# Autodesk Inventor assembly: ASY дренаж угольные
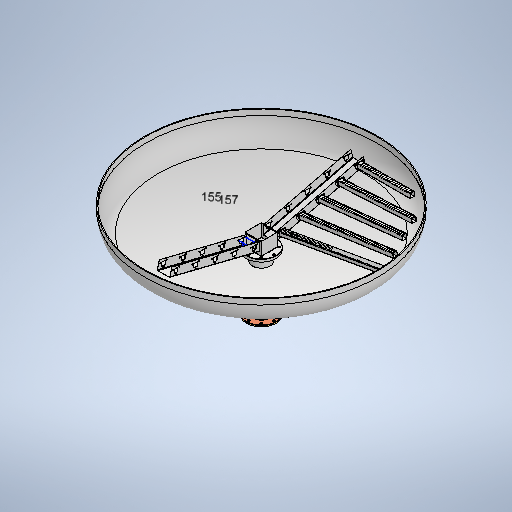
[picture p0: Inventor's stored thumbnail of the model, 512x512]
Saved by Autodesk Inventor 2025 (Build 290162010, 162A)
## iProperties
Created: 2024-12-09
Part Number: ASY дренаж угольные
Document SubType Name: Assembly
Designer: user
Author: user
## Documents named in this file (21)
- C:\Users\pokla\Documents\Inventor\Отстойник осветлитель\Manturovo_Se-clar-Gleb\Дренаж на угольные\ASY дренаж угольные.iam
- C:\Users\pokla\Documents\Inventor\Отстойник осветлитель\Manturovo_Se-clar-Gleb\Дренаж на угольные\Main filter Flange.ipt
- C:\Users\pokla\Documents\Inventor\Отстойник осветлитель\Manturovo_Se-clar-Gleb\Дренаж на угольные\drain flange.ipt
- C:\Users\pokla\Documents\Inventor\Отстойник осветлитель\Manturovo_Se-clar-Gleb\Дренаж на угольные\Part9.ipt
- C:\Users\pokla\Documents\Inventor\Отстойник осветлитель\Manturovo_Se-clar-Gleb\Дренаж на угольные\drain bottom plate.ipt
- C:\Users\pokla\Documents\Inventor\Отстойник осветлитель\Manturovo_Se-clar-Gleb\Дренаж на угольные\drain wall with flange.ipt
- C:\Users\user\YandexDisk-badmisterfox\домашниий пк\Inventor\Manturovo\Content Center Files\en-US\DIN 933\DIN 933 - M12  x 35.ipt
- C:\Users\pokla\Documents\Inventor\Отстойник осветлитель\Manturovo_Se-clar-Gleb\Дренаж на угольные\drain cup.ipt
- C:\Users\pokla\Documents\Inventor\Отстойник осветлитель\Manturovo_Se-clar-Gleb\Дренаж на угольные\Фильтр напорный угольный 30 куб час.ipt
- C:\Users\pokla\Documents\Inventor\Отстойник осветлитель\Manturovo_Se-clar-Gleb\Дренаж на угольные\MNT-CDF-301 beam 1.ipt
- C:\Users\pokla\Documents\Inventor\Отстойник осветлитель\Manturovo_Se-clar-Gleb\Дренаж на угольные\MNT-CDF-401 roof 1.ipt
- C:\Users\pokla\Documents\Inventor\Отстойник осветлитель\Manturovo_Se-clar-Gleb\Дренаж на угольные\MNT-CDF-501 box.ipt
- C:\Users\pokla\Documents\Inventor\Отстойник осветлитель\Manturovo_Se-clar-Gleb\Дренаж на угольные\MNT-CDF-502 tube.ipt
- C:\Users\pokla\Documents\Inventor\Отстойник осветлитель\Manturovo_Se-clar-Gleb\Дренаж на угольные\MNT-CDF-503  main tube 1.ipt
- C:\Users\user\YandexDisk-badmisterfox\домашниий пк\Inventor\Manturovo\Content Center Files\en-US\DIN 933\DIN 933 - M8  x 20.ipt
- C:\Users\pokla\Documents\Inventor\Отстойник осветлитель\Manturovo_Se-clar-Gleb\Дренаж на угольные\MNT-CDF-504 small tube flange.ipt
- C:\Users\pokla\Documents\Inventor\Отстойник осветлитель\Manturovo_Se-clar-Gleb\Дренаж на угольные\MNT-CDF-315 beam 5.ipt
- C:\Users\pokla\Documents\Inventor\Отстойник осветлитель\Manturovo_Se-clar-Gleb\Дренаж на угольные\MNT-CDF-312 beam 2.ipt
- C:\Users\pokla\Documents\Inventor\Отстойник осветлитель\Manturovo_Se-clar-Gleb\Дренаж на угольные\MNT-CDF-313 beam 3.ipt
- C:\Users\pokla\Documents\Inventor\Отстойник осветлитель\Manturovo_Se-clar-Gleb\Дренаж на угольные\MNT-CDF-314 beam 4.ipt
- C:\Users\pokla\Documents\Inventor\NDM-VOS_powder_hopper\Workspaces\Workspace\Cone\MNT-CDF-601 CAP.ipt
## Components (39 placed, 20 different names)
1. Main filter Flange.ipt:1 — Rigid:1
2. drain flange.ipt:1 — Rigid:1, Rigid:7
3. Part9.ipt:1 — Rigid:4, Rigid:7
4. drain bottom plate.ipt:1 — Rigid:4, Rigid:5, Rigid:6
5. drain wall with flange:1 — Rigid:3, Rigid:6, Mate:2, Flush:1, Rotational:2, Rotational:3, Rotational:4
6. DIN 933 - replaced by DIN EN 24017 M12  x 35:1 — Rigid:3
7. drain wall with flange:2 — Rigid:5, Mate:1, Rotational:1
8. DIN 933 - replaced by DIN EN 24017 M12  x 35:2 — Rotational:1
9. DIN 933 - replaced by DIN EN 24017 M12  x 35:3 — Rotational:3
10. Part1:3 — Mate:1, Mate:2, Flush:1, Rotational:5, Rotational:6
11. DIN 933 - replaced by DIN EN 24017 M12  x 35:4 — Rotational:2
12. DIN 933 - replaced by DIN EN 24017 M12  x 35:5 — Rotational:4
13. DIN 933 - replaced by DIN EN 24017 M12  x 35:6 — Rotational:6
14. DIN 933 - replaced by DIN EN 24017 M12  x 35:7 — Rotational:5
15. Фильтр напорный угольный 30 куб час:1 — Mate:4, Flush:3, Flush:4, Rigid:12
16. MNT-CDF-301 beam 1:1 — Flush:2, Mate:8, Flush:9, Rigid:22
17. MNT-CDF-401 roof 1:1 — Flush:2, Mate:8, Flush:9
18. MNT-CDF-501 box:1 — Rotational:9, Flush:8, Mate:9, Mate:10, Rotational:10, Rotational:11
19. drain flange:2 — Rigid:12, Mate:5
20. MNT-CDF-502 tube:4 — Rotational:11
21. MNT-CDF-502 tube:3 — Rotational:10
22. MNT-CDF-502 tube:2 — Rotational:9
23. MNT-CDF-503  main tube 1:1 — Rigid:14, Rigid:15
24. MNT-CDF-503  main tube 1:2 — Rigid:14, Mate:5, Mate:6, Mate:9, Mate:10
25. MNT-CDF-501 box:2 — Rigid:15, Rigid:18, Rigid:19, Rigid:20, Rigid:23, Rigid:24, Rigid:25
26. DIN 933 - replaced by DIN EN 24017 M8  x 20:1 — Rotational:12
27. Part1:4 — Rigid:18, Rigid:22, Rotational:12, Rotational:13, Rotational:14
28. MNT-CDF-502 tube:5 — Rigid:19
29. MNT-CDF-315 beam 5:1 — Rigid:21
30. Part1:5 — Rigid:20, Rigid:21
31. DIN 933 - replaced by DIN EN 24017 M8  x 20:2 — Rotational:14
32. DIN 933 - replaced by DIN EN 24017 M8  x 20:3 — Rotational:13
33. MNT-CDF-312 beam 2:1 — Rigid:26
34. Part1:6 — Rigid:23, Rigid:26
35. Part1:7 — Rigid:24, Rigid:27
36. Part1:8 — Rigid:25, Rigid:28
37. MNT-CDF-313 beam 3:1 — Rigid:27
38. MNT-CDF-314 beam 4:1 — Rigid:28
39. MNT-CDF-601 CAP:1
## Relationships (46: WeldJoint 20, RevoluteJoint 12, Mate 8, Flush 6)
- Rigid:1 [WeldJoint]: Main filter Flange.ipt:1 ↔ drain flange.ipt:1
- Rigid:3 [WeldJoint]: drain wall with flange:1 ↔ DIN 933 - replaced by DIN EN 24017 M12  x 35:1
- Rigid:4 [WeldJoint]: Part9.ipt:1 ↔ drain bottom plate.ipt:1
- Rigid:5 [WeldJoint]: drain bottom plate.ipt:1 ↔ drain wall with flange:2
- Rigid:6 [WeldJoint]: drain bottom plate.ipt:1 ↔ drain wall with flange:1
- Rotational:1 [RevoluteJoint]: drain wall with flange:2 ↔ DIN 933 - replaced by DIN EN 24017 M12  x 35:2
- Rigid:7 [WeldJoint]: drain flange.ipt:1 ↔ Part9.ipt:1
- Mate:1: drain wall with flange:2 ↔ Part1:3
- Mate:2: drain wall with flange:1 ↔ Part1:3
- Flush:1: drain wall with flange:1 ↔ Part1:3
- Rotational:2 [RevoluteJoint]: drain wall with flange:1 ↔ DIN 933 - replaced by DIN EN 24017 M12  x 35:4
- Rotational:3 [RevoluteJoint]: drain wall with flange:1 ↔ DIN 933 - replaced by DIN EN 24017 M12  x 35:3
- Rotational:4 [RevoluteJoint]: drain wall with flange:1 ↔ DIN 933 - replaced by DIN EN 24017 M12  x 35:5
- Rotational:5 [RevoluteJoint]: Part1:3 ↔ DIN 933 - replaced by DIN EN 24017 M12  x 35:7
- Rotational:6 [RevoluteJoint]: Part1:3 ↔ DIN 933 - replaced by DIN EN 24017 M12  x 35:6
- Flush:2: MNT-CDF-301 beam 1:1 ↔ MNT-CDF-401 roof 1:1
- Mate:4: Фильтр напорный угольный 30 куб час:1
- Flush:3: Фильтр напорный угольный 30 куб час:1
- Flush:4: Фильтр напорный угольный 30 куб час:1
- Rigid:12 [WeldJoint]: Фильтр напорный угольный 30 куб час:1 ↔ drain flange:2
- Rotational:9 [RevoluteJoint]: MNT-CDF-501 box:1 ↔ MNT-CDF-502 tube:2
- Rigid:14 [WeldJoint]: MNT-CDF-503  main tube 1:1 ↔ MNT-CDF-503  main tube 1:2
- Mate:5: drain flange:2 ↔ MNT-CDF-503  main tube 1:2
- Mate:6: MNT-CDF-503  main tube 1:2
- Flush:8: MNT-CDF-501 box:1
- Mate:8: MNT-CDF-301 beam 1:1 ↔ MNT-CDF-401 roof 1:1
- Mate:9: MNT-CDF-501 box:1 ↔ MNT-CDF-503  main tube 1:2
- Mate:10: MNT-CDF-501 box:1 ↔ MNT-CDF-503  main tube 1:2
- Rigid:15 [WeldJoint]: MNT-CDF-503  main tube 1:1 ↔ MNT-CDF-501 box:2
- Flush:9: MNT-CDF-301 beam 1:1 ↔ MNT-CDF-401 roof 1:1
- Rotational:10 [RevoluteJoint]: MNT-CDF-501 box:1 ↔ MNT-CDF-502 tube:3
- Rotational:11 [RevoluteJoint]: MNT-CDF-501 box:1 ↔ MNT-CDF-502 tube:4
- Rigid:18 [WeldJoint]: MNT-CDF-501 box:2 ↔ Part1:4
- Rigid:19 [WeldJoint]: MNT-CDF-501 box:2 ↔ MNT-CDF-502 tube:5
- Rigid:20 [WeldJoint]: MNT-CDF-501 box:2 ↔ Part1:5
- Rigid:21 [WeldJoint]: MNT-CDF-315 beam 5:1 ↔ Part1:5
- Rigid:22 [WeldJoint]: MNT-CDF-301 beam 1:1 ↔ Part1:4
- Rotational:12 [RevoluteJoint]: DIN 933 - replaced by DIN EN 24017 M8  x 20:1 ↔ Part1:4
- Rotational:13 [RevoluteJoint]: Part1:4 ↔ DIN 933 - replaced by DIN EN 24017 M8  x 20:3
- Rotational:14 [RevoluteJoint]: Part1:4 ↔ DIN 933 - replaced by DIN EN 24017 M8  x 20:2
- Rigid:23 [WeldJoint]: MNT-CDF-501 box:2 ↔ Part1:6
- Rigid:24 [WeldJoint]: MNT-CDF-501 box:2 ↔ Part1:7
- Rigid:25 [WeldJoint]: MNT-CDF-501 box:2 ↔ Part1:8
- Rigid:26 [WeldJoint]: MNT-CDF-312 beam 2:1 ↔ Part1:6
- Rigid:27 [WeldJoint]: Part1:7 ↔ MNT-CDF-313 beam 3:1
- Rigid:28 [WeldJoint]: Part1:8 ↔ MNT-CDF-314 beam 4:1
